# Autodesk Inventor assembly: 000.005.004 - Поворот сгиба кисти СБ
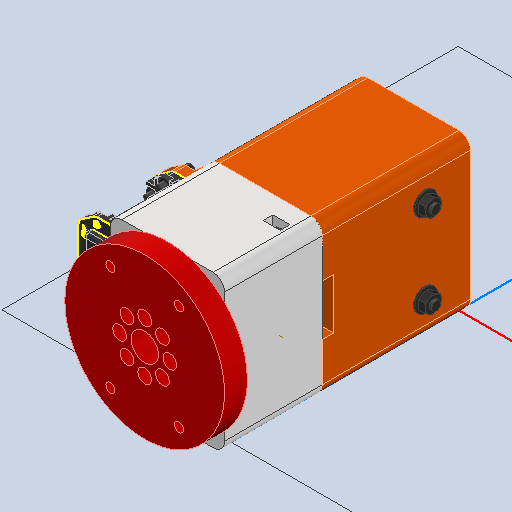
[picture p0: Inventor's stored thumbnail of the model, 512x512]
Saved by Autodesk Inventor 2022 (Build 260153000, 153)
## iProperties
Created: 2022-12-17
Part Number: 000.005.004 - Поворот сгиба кисти СБ
Document SubType Name: Assembly
Designer: Petrov Ivan
Mass: 309.284 g
Surface Area: 856.638 cm^2
Volume: 287.74 cm^3
Density: 1.07487 g/cm^3
Author: Petrov Ivan
## Documents named in this file (16)
- C:\Users\Ivan Petrov\Documents\GitHub\OmniBot\design\000.005.004 - Поворот сгиба кисти СБ.iam
- C:\Users\Ivan Petrov\Documents\GitHub\OmniBot\design\000.005.004.001 - Основание.ipt
- C:\Users\Ivan Petrov\Documents\GitHub\OmniBot\design\standart_components\dynamixels\mx-64\MX-64T.iam
- C:\Users\Ivan Petrov\Documents\GitHub\OmniBot\design\Content Center Files\R2022\ru-RU\BS EN 24035\ISO 4035 - M2.5BS EN.ipt
- C:\Users\Ivan Petrov\Documents\GitHub\OmniBot\design\Content Center Files\R2022\ru-RU\ISO 4762(1)\DIN EN ISO 4762 - M2.5 x 12.ipt
- C:\Users\Ivan Petrov\Documents\GitHub\OmniBot\design\Content Center Files\R2022\ru-RU\ISO 4762(1)\DIN EN ISO 4762 - M2.5 x 25.ipt
- C:\Users\Ivan Petrov\Documents\GitHub\OmniBot\design\000.005.004.002 - Скоба.ipt
- C:\Users\Ivan Petrov\Documents\GitHub\OmniBot\design\Content Center Files\R2022\ru-RU\ISO 4762(1)\DIN EN ISO 4762 - M2.5 x 10.ipt
- C:\Users\Ivan Petrov\Documents\GitHub\OmniBot\design\000.005.004.003 - Поворотный диск.ipt
- C:\Users\Ivan Petrov\Documents\GitHub\OmniBot\design\Content Center Files\R2022\ru-RU\ISO 4762(1)\DIN EN ISO 4762 - M2.5 x 6.ipt
- C:\Users\Ivan Petrov\Documents\GitHub\OmniBot\design\Content Center Files\R2022\ru-RU\ISO 4762(1)\DIN EN ISO 4762 - M2.5 x 16.ipt
- C:\Users\Ivan Petrov\Documents\GitHub\OmniBot\design\Content Center Files\ru-RU\DIN 976-1 A\DIN 976-1 - M4 x 60 - A.ipt
- C:\Users\Ivan Petrov\Documents\GitHub\OmniBot\design\Content Center Files\ru-RU\CNS 4309\CNS 4309 - 4,5 x 10 A.ipt
- C:\Users\Ivan Petrov\Documents\GitHub\OmniBot\design\Content Center Files\ru-RU\AS 1112 (2)\AS 1112 - M4  Тип 5.ipt
- C:\Users\Ivan Petrov\Documents\GitHub\OmniBot\design\Content Center Files\ru-RU\AS 1112 (2)\AS 1112 - M4  Тип 10.ipt
- C:\Users\Ivan Petrov\Documents\GitHub\OmniBot\design\Content Center Files\ru-RU\CSN 02 1143  B\CSN 02 1143 - M4 x 0,7 x 25(2).ipt
## Components (50 placed, 15 different names)
1. 000.005.004.001 - Основание:1 — Угол:3, Совмещение:5, Совмещение:6, Вставка:9, Вставка:10, Вставка:11, Вставка:12, Вставка:14, Вставка:15, Заподлицо:1, Заподлицо:2, Совмещение:13, Вставка:33, Вставка:34, Совмещение:14, Совмещение:15, Заподлицо:3, Заподлицо:4, Вставка:35, Вставка:36, Вставка:37, Вставка:38, Вставка:47, Вставка:48, Вставка:49, Вставка:50
2. MX-64T:1 [sub-assembly] — Угол:3, Совмещение:5, Совмещение:6, Вставка:1, Вставка:2, Вставка:3, Вставка:4, Вставка:5, Вставка:6, Вставка:7, Вставка:8, Совмещение:9, Совмещение:10, Совмещение:11
3. 000.005.004.002 - Скоба:1 — Заподлицо:1, Заподлицо:2, Вставка:17, Вставка:18, Вставка:19, Вставка:20, Совмещение:13, Вставка:43, Вставка:44, Вставка:45, Вставка:46
4. 000.005.004.003 - Поворотный диск:1 — Совмещение:9, Совмещение:10, Совмещение:11, Вставка:21, Вставка:22, Вставка:23, Вставка:24, Вставка:25, Вставка:26, Вставка:27, Вставка:28
5. DIN EN ISO 4762 M2,5 x 16:1 — Вставка:33
6. DIN EN ISO 4762 M2,5 x 16:2 — Вставка:34
7. DIN 976-1 A M4 x 60:1 — Совмещение:14, Заподлицо:3
8. DIN 976-1 A M4 x 60:2 — Совмещение:15, Заподлицо:4
9. CNS 4309 4,5 A:1 — Вставка:35, Вставка:42
10. CNS 4309 4,5 A:2 — Вставка:36, Вставка:41
11. CNS 4309 4,5 A:3 — Вставка:37, Вставка:39
12. CNS 4309 4,5 A:4 — Вставка:38, Вставка:40
13. AS 1112 (2) - метрическая M4  Тип 5:1 — Вставка:39
14. AS 1112 (2) - метрическая M4  Тип 5:2 — Вставка:40
15. AS 1112 (2) - метрическая M4  Тип 5:3 — Вставка:41
16. AS 1112 (2) - метрическая M4  Тип 5:4 — Вставка:42
17. AS 1112 (2) - метрическая M4  Тип 10:1 — Вставка:43
18. AS 1112 (2) - метрическая M4  Тип 10:2 — Вставка:44
19. AS 1112 (2) - метрическая M4  Тип 10:3 — Вставка:45
20. AS 1112 (2) - метрическая M4  Тип 10:4 — Вставка:46
21. CSN 02 1143 B M4 x 25:1 — Вставка:47
22. CSN 02 1143 B M4 x 25:2 — Вставка:48
23. CSN 02 1143 B M4 x 25:3 — Вставка:49
24. CSN 02 1143 B M4 x 25:4 — Вставка:50
25. DIN EN ISO 4762 M2,5 x 10:1 — Вставка:17
26. DIN EN ISO 4762 M2,5 x 10:2 — Вставка:18
27. DIN EN ISO 4762 M2,5 x 10:3 — Вставка:19
28. DIN EN ISO 4762 M2,5 x 10:4 — Вставка:20
29. BS EN 24035 - метрическая M2,5:1 — Вставка:1
30. BS EN 24035 - метрическая M2,5:2 — Вставка:2
31. BS EN 24035 - метрическая M2,5:3 — Вставка:3
32. BS EN 24035 - метрическая M2,5:4 — Вставка:4
33. BS EN 24035 - метрическая M2,5:5 — Вставка:5
34. BS EN 24035 - метрическая M2,5:6 — Вставка:6
35. BS EN 24035 - метрическая M2,5:7 — Вставка:7
36. BS EN 24035 - метрическая M2,5:8 — Вставка:8
37. DIN EN ISO 4762 M2,5 x 12:1 — Вставка:9
38. DIN EN ISO 4762 M2,5 x 12:2 — Вставка:10
39. DIN EN ISO 4762 M2,5 x 12:3 — Вставка:11
40. DIN EN ISO 4762 M2,5 x 12:4 — Вставка:12
41. DIN EN ISO 4762 M2,5 x 25:2 — Вставка:14
42. DIN EN ISO 4762 M2,5 x 25:3 — Вставка:15
43. DIN EN ISO 4762 M2,5 x 6:1 — Вставка:21
44. DIN EN ISO 4762 M2,5 x 6:2 — Вставка:22
45. DIN EN ISO 4762 M2,5 x 6:3 — Вставка:23
46. DIN EN ISO 4762 M2,5 x 6:4 — Вставка:24
47. DIN EN ISO 4762 M2,5 x 6:5 — Вставка:25
48. DIN EN ISO 4762 M2,5 x 6:6 — Вставка:26
49. DIN EN ISO 4762 M2,5 x 6:7 — Вставка:27
50. DIN EN ISO 4762 M2,5 x 6:8 — Вставка:28
## Relationships (57: Insert 44, Mate 8, Flush 4, Angle 1)
- Угол:3 [Angle] (-90 deg): 000.005.004.001 - Основание:1 ↔ MX-64T:1
- Совмещение:5 [Mate]: 000.005.004.001 - Основание:1 ↔ MX-64T:1
- Совмещение:6 [Mate]: 000.005.004.001 - Основание:1 ↔ MX-64T:1
- Вставка:1 [Insert]: MX-64T:1 ↔ BS EN 24035 - метрическая M2,5:1
- Вставка:2 [Insert]: MX-64T:1 ↔ BS EN 24035 - метрическая M2,5:2
- Вставка:3 [Insert]: MX-64T:1 ↔ BS EN 24035 - метрическая M2,5:3
- Вставка:4 [Insert]: MX-64T:1 ↔ BS EN 24035 - метрическая M2,5:4
- Вставка:5 [Insert]: MX-64T:1 ↔ BS EN 24035 - метрическая M2,5:5
- Вставка:6 [Insert]: MX-64T:1 ↔ BS EN 24035 - метрическая M2,5:6
- Вставка:7 [Insert]: MX-64T:1 ↔ BS EN 24035 - метрическая M2,5:7
- Вставка:8 [Insert]: MX-64T:1 ↔ BS EN 24035 - метрическая M2,5:8
- Вставка:9 [Insert]: 000.005.004.001 - Основание:1 ↔ DIN EN ISO 4762 M2,5 x 12:1
- Вставка:10 [Insert]: 000.005.004.001 - Основание:1 ↔ DIN EN ISO 4762 M2,5 x 12:2
- Вставка:11 [Insert]: 000.005.004.001 - Основание:1 ↔ DIN EN ISO 4762 M2,5 x 12:3
- Вставка:12 [Insert]: 000.005.004.001 - Основание:1 ↔ DIN EN ISO 4762 M2,5 x 12:4
- Вставка:14 [Insert]: 000.005.004.001 - Основание:1 ↔ DIN EN ISO 4762 M2,5 x 25:2
- Вставка:15 [Insert]: 000.005.004.001 - Основание:1 ↔ DIN EN ISO 4762 M2,5 x 25:3
- Заподлицо:1 [Flush]: 000.005.004.001 - Основание:1 ↔ 000.005.004.002 - Скоба:1
- Заподлицо:2 [Flush]: 000.005.004.001 - Основание:1 ↔ 000.005.004.002 - Скоба:1
- Вставка:17 [Insert]: 000.005.004.002 - Скоба:1 ↔ DIN EN ISO 4762 M2,5 x 10:1
- Вставка:18 [Insert]: 000.005.004.002 - Скоба:1 ↔ DIN EN ISO 4762 M2,5 x 10:2
- Вставка:19 [Insert]: 000.005.004.002 - Скоба:1 ↔ DIN EN ISO 4762 M2,5 x 10:3
- Вставка:20 [Insert]: 000.005.004.002 - Скоба:1 ↔ DIN EN ISO 4762 M2,5 x 10:4
- Совмещение:9 [Mate]: MX-64T:1 ↔ 000.005.004.003 - Поворотный диск:1
- Совмещение:10 [Mate]: MX-64T:1 ↔ 000.005.004.003 - Поворотный диск:1
- Совмещение:11 [Mate]: MX-64T:1 ↔ 000.005.004.003 - Поворотный диск:1
- Вставка:21 [Insert]: 000.005.004.003 - Поворотный диск:1 ↔ DIN EN ISO 4762 M2,5 x 6:1
- Вставка:22 [Insert]: 000.005.004.003 - Поворотный диск:1 ↔ DIN EN ISO 4762 M2,5 x 6:2
- Вставка:23 [Insert]: 000.005.004.003 - Поворотный диск:1 ↔ DIN EN ISO 4762 M2,5 x 6:3
- Вставка:24 [Insert]: 000.005.004.003 - Поворотный диск:1 ↔ DIN EN ISO 4762 M2,5 x 6:4
- Вставка:25 [Insert]: 000.005.004.003 - Поворотный диск:1 ↔ DIN EN ISO 4762 M2,5 x 6:5
- Вставка:26 [Insert]: 000.005.004.003 - Поворотный диск:1 ↔ DIN EN ISO 4762 M2,5 x 6:6
- Вставка:27 [Insert]: 000.005.004.003 - Поворотный диск:1 ↔ DIN EN ISO 4762 M2,5 x 6:7
- Вставка:28 [Insert]: 000.005.004.003 - Поворотный диск:1 ↔ DIN EN ISO 4762 M2,5 x 6:8
- Совмещение:13 [Mate]: 000.005.004.001 - Основание:1 ↔ 000.005.004.002 - Скоба:1
- Вставка:33 [Insert]: 000.005.004.001 - Основание:1 ↔ DIN EN ISO 4762 M2,5 x 16:1
- Вставка:34 [Insert]: 000.005.004.001 - Основание:1 ↔ DIN EN ISO 4762 M2,5 x 16:2
- Совмещение:14 [Mate]: 000.005.004.001 - Основание:1 ↔ DIN 976-1 A M4 x 60:1
- Совмещение:15 [Mate]: 000.005.004.001 - Основание:1 ↔ DIN 976-1 A M4 x 60:2
- Заподлицо:3 [Flush] (-5 mm): 000.005.004.001 - Основание:1 ↔ DIN 976-1 A M4 x 60:1
- Заподлицо:4 [Flush] (-5 mm): 000.005.004.001 - Основание:1 ↔ DIN 976-1 A M4 x 60:2
- Вставка:35 [Insert]: 000.005.004.001 - Основание:1 ↔ CNS 4309 4,5 A:1
- Вставка:36 [Insert]: 000.005.004.001 - Основание:1 ↔ CNS 4309 4,5 A:2
- Вставка:37 [Insert]: 000.005.004.001 - Основание:1 ↔ CNS 4309 4,5 A:3
- Вставка:38 [Insert]: 000.005.004.001 - Основание:1 ↔ CNS 4309 4,5 A:4
- Вставка:39 [Insert]: CNS 4309 4,5 A:3 ↔ AS 1112 (2) - метрическая M4  Тип 5:1
- Вставка:40 [Insert]: CNS 4309 4,5 A:4 ↔ AS 1112 (2) - метрическая M4  Тип 5:2
- Вставка:41 [Insert]: CNS 4309 4,5 A:2 ↔ AS 1112 (2) - метрическая M4  Тип 5:3
- Вставка:42 [Insert]: CNS 4309 4,5 A:1 ↔ AS 1112 (2) - метрическая M4  Тип 5:4
- Вставка:43 [Insert]: 000.005.004.002 - Скоба:1 ↔ AS 1112 (2) - метрическая M4  Тип 10:1
- Вставка:44 [Insert]: 000.005.004.002 - Скоба:1 ↔ AS 1112 (2) - метрическая M4  Тип 10:2
- Вставка:45 [Insert]: 000.005.004.002 - Скоба:1 ↔ AS 1112 (2) - метрическая M4  Тип 10:3
- Вставка:46 [Insert]: 000.005.004.002 - Скоба:1 ↔ AS 1112 (2) - метрическая M4  Тип 10:4
- Вставка:47 [Insert]: 000.005.004.001 - Основание:1 ↔ CSN 02 1143 B M4 x 25:1
- Вставка:48 [Insert]: 000.005.004.001 - Основание:1 ↔ CSN 02 1143 B M4 x 25:2
- Вставка:49 [Insert]: 000.005.004.001 - Основание:1 ↔ CSN 02 1143 B M4 x 25:3
- Вставка:50 [Insert]: 000.005.004.001 - Основание:1 ↔ CSN 02 1143 B M4 x 25:4
